# Autodesk Inventor assembly: Joes_Robot
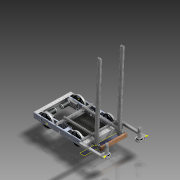
[picture p0: Inventor's stored thumbnail of the model, 180x180]
Saved by Autodesk Inventor 2015 (Build 190159000, 159)
## iProperties
Created: 2015-01-23
Part Number: Joes_Robot
Document SubType Name: Assembly
Designer: 55221
Author: 55221
## Documents named in this file (27)
- C:\Users\Kingbob26\Documents\GitHub\2015CAD\Misc\Joes_Robot.iam
- C:\Users\Kingbob26\Documents\GitHub\2015CAD\wheelBase\Outside Sheet Square.ipt
- C:\Users\Kingbob26\Documents\GitHub\2015CAD\wheelBase\2x3 Hole Bracket.ipt
- C:\Users\Kingbob26\Documents\GitHub\2015CAD\wheelBase\Inside Sheet Square.ipt
- C:\Users\Kingbob26\Documents\GitHub\2015CAD\wheelBase\TB Output Shaft Hex L-Base 2.ipt
- C:\Users\Kingbob26\Documents\Inventor\Sheet Metal Front-Back.ipt.ipt
- C:\Users\Kingbob26\Documents\GitHub\2015CAD\actualWheelBase\Drive Base\Parts\simpleGBFull.iam
- C:\Users\Kingbob26\Documents\GitHub\2015CAD\actualWheelBase\Drive Base\Parts\8inDriveWheel.iam
- C:\Users\Kingbob26\Documents\GitHub\2015CAD\wheelBase\Hex Bearing.ipt
- C:\Users\Kingbob26\Documents\GitHub\2015CAD\Motion\alignmentWheelsBar.ipt
- C:\Users\Kingbob26\Documents\GitHub\2015CAD\Motion\alignmentWheelsBarP2.ipt
- C:\Users\Kingbob26\Documents\GitHub\2015CAD\Motion\alignmentWheelsMotor.ipt
- C:\Users\Kingbob26\Documents\GitHub\2015CAD\wheelBase\4in 2013 Hub.ipt
- C:\Users\Kingbob26\Documents\GitHub\2015CAD\wheelBase\4 in tread.ipt
- C:\Users\Kingbob26\Documents\GitHub\2015CAD\wheelBase\keyStoneHub10mm.ipt
- C:\Users\Kingbob26\Documents\GitHub\2015CAD\Misc\Imported Components\T-slottedFraming\T-slottedFraming.ipt
- C:\Users\Kingbob26\Documents\GitHub\2015CAD\Motion\GuidanceShaft.ipt
- C:\Users\Kingbob26\Documents\GitHub\2015CAD\Motion\Roller.ipt
- C:\Users\Kingbob26\Documents\GitHub\2015CAD\Misc\Imported Components\90framing\90framing.ipt
- C:\Users\Kingbob26\Documents\GitHub\2015CAD\Misc\Imported Components\specialScrews\specialScrews.ipt
- C:\Users\Kingbob26\Documents\GitHub\2015CAD\Misc\T-slottedFramingCustomLength25.5.ipt
- C:\Users\Kingbob26\Documents\GitHub\2015CAD\Misc\Imported Components\90degreeAngleBracket\90degreeAngleBracket.ipt
- C:\Users\Kingbob26\Documents\GitHub\2015CAD\Misc\liftingMechanismPlate.ipt
- C:\Users\Kingbob26\Documents\GitHub\2015CAD\Misc\Imported Components\1x1tCap\1x1tCap.ipt
- C:\Users\Kingbob26\Documents\GitHub\2015CAD\Misc\Crossbar.ipt
- C:\Users\Kingbob26\Documents\GitHub\2015CAD\Motion\lBracketForLiftingBar.ipt
- Sheet Metal Front-Back.ipt
## Components (60 placed, 25 different names)
1. Outside Sheet Square:1 — Mate:124, Mate:181, Mate:183, Mate:189, Mate:206, Mate:207, Mate:245, Mate:246, Mate:335
2. 2x3 Hole Bracket:2 — Mate:116, Mate:117, Mate:118, Mate:124, Mate:335
3. Inside Sheet Square:1 — Mate:116, Mate:117, Mate:118, Mate:150, Mate:182, Mate:184, Mate:188, Mate:204, Mate:205, Angle:9, Flush:2
4. Inside Sheet Square:2 — Mate:131, Mate:132, Mate:134, Mate:180, Mate:185, Insert:1, Angle:5, Mate:201, Mate:202, Mate:203, Flush:3, Mate:316, Mate:317, Mate:318
5. Outside Sheet Square:2 — Mate:133, Mate:178, Mate:179, Mate:186, Mate:187, Mate:208, Mate:209, Mate:247, Mate:248, Mate:263, Mate:281, Mate:298, Mate:300
6. 2x3 Hole Bracket:3 — Mate:131, Mate:132, Mate:133, Mate:134, Mate:281
7. TB Output Shaft Hex L-Base 2:3 — Mate:150, Angle:8
8. Sheet Metal Front-Back.ipt:1 — Mate:178, Mate:179, Mate:180, Mate:181, Mate:182, Mate:183, Mate:184, Angle:17, Mate:278, Mate:282, Flush:4, Mate:299, Flush:8, Mate:303, Flush:19, Flush:22
9. Sheet Metal Front-Back.ipt:2 — Mate:185, Mate:186, Mate:187, Mate:188, Mate:189, Mate:263
10. simpleGBFull:1 [sub-assembly] — Angle:9
11. 8inDriveWheel:1 [sub-assembly]
12. simpleGBFull:2 [sub-assembly] — Insert:1, Angle:5, Mate:198, Mate:199
13. TB Output Shaft Hex L-Base 2:4 — Mate:198, Mate:199, Mate:200, Angle:6, Angle:7
14. 8inDriveWheel:4 [sub-assembly] — Mate:200, Angle:6, Mate:201
15. 8inDriveWheel:5 [sub-assembly] — Mate:202, Mate:203
16. 8inDriveWheel:6 [sub-assembly] — Mate:204, Mate:205
17. Hex Bearing:1 — Mate:206, Mate:207, Angle:8
18. Hex Bearing:2 — Mate:208, Mate:209, Angle:7
19. alignmentWheelsBar:1 — Mate:217, Mate:218, Mate:245, Mate:246
20. alignmentWheelsBar:2 — Mate:243, Mate:244, Mate:247, Mate:248
21. alignmentWheelsBarP2:1 — Mate:243, Mate:244, Insert:4, Mate:251
22. alignmentWheelsBarP2:2 — Mate:217, Mate:218, Insert:5, Mate:249
23. alignmentWheelsMotor:1 — Angle:10, Mate:249, Mate:250
24. alignmentWheelsMotor:2 — Angle:11, Mate:251, Mate:252
25. 4in 2013 Hub:1 — Insert:3, Mate:237, Mate:238, Mate:239
26. 4in 2013 Hub:2 — Insert:2, Mate:240, Mate:241, Mate:242
27. 4 in tread:1 — Insert:3
28. 4 in tread:2 — Insert:2
29. keyStoneHub10mm:1 — Mate:237, Mate:238, Mate:239, Angle:10, Insert:5, Mate:250
30. keyStoneHub10mm:2 — Mate:240, Mate:241, Mate:242, Angle:11, Insert:4, Mate:252
31. T-slottedFraming:1 — Flush:4, Mate:291, Mate:296, Mate:298, Mate:299, Flush:9, Mate:301, Mate:305, Mate:306, Mate:308, Flush:18
32. GuidanceShaft:1 — Flush:2, Angle:17, Mate:278, Mate:279, Mate:280, Angle:20, Angle:21, Angle:22, Angle:28, Angle:29, Mate:321, Mate:322
33. GuidanceShaft:2 — Flush:3, Mate:271, Mate:282
34. Roller:1 — Angle:28, Angle:29, Mate:321, Mate:322, Mate:324, Mate:325, Mate:326, Angle:30, Mate:329, Flush:20, Flush:21
35. 90framing:1 — Mate:271, Insert:6, Angle:13, Angle:14, Insert:7, Mate:320, Flush:17
36. specialScrews:1 — Insert:6, Angle:13
37. specialScrews:3 — Angle:14, Insert:7
38. 90framing:2 — Mate:279, Mate:280, Insert:8, Insert:9, Mate:319, Flush:16
39. T-slottedFraming:2 — Mate:288, Mate:292, Flush:5, Mate:294, Mate:300, Flush:8, Mate:303, Angle:23, Mate:304, Flush:11, Mate:310, Mate:312
40. specialScrews:4 — Angle:20, Insert:8
41. specialScrews:5 — Angle:21, Insert:9
42. T-slottedFramingCustomLength25.5:1 — Mate:288, Angle:22, Mate:291, Flush:5, Mate:293, Flush:6, Mate:295, Mate:297, Mate:302, Mate:320, Flush:17, Angle:24, Insert:10, Angle:26, Insert:12, Flush:18
43. T-slottedFramingCustomLength25.5:2 — Angle:23, Mate:304, Flush:11, Mate:305, Mate:307, Mate:309, Mate:311, Mate:313, Mate:319, Flush:16, Angle:25, Insert:11, Angle:27, Insert:13, Flush:19
44. 90degreeAngleBracket:1 — Mate:294, Mate:295, Flush:7, Flush:14
45. 90degreeAngleBracket:2 — Mate:301, Mate:302, Flush:10, Flush:12
46. 90degreeAngleBracket:3 — Mate:296, Mate:297, Flush:9, Flush:10, Flush:13
47. 90degreeAngleBracket:4 — Mate:292, Mate:293, Flush:6, Flush:7
48. 90degreeAngleBracket:5 — Mate:308, Mate:309, Flush:13
49. 90degreeAngleBracket:6 — Mate:306, Mate:307, Flush:12
50. 90degreeAngleBracket:7 — Mate:312, Mate:313, Flush:15
51. 90degreeAngleBracket:8 — Mate:310, Mate:311, Flush:14, Flush:15
52. liftingMechanismPlate:1 — Mate:316, Mate:317, Mate:318
53. 1x1tCap:1 — Angle:27, Insert:13
54. 1x1tCap:2 — Angle:26, Insert:12
55. 1x1tCap:3 — Angle:25, Insert:11
56. 1x1tCap:4 — Angle:24, Insert:10
57. Crossbar:1 — Mate:328, Mate:333, Mate:334
58. Roller:2 — Angle:30, Mate:329, Flush:20, Flush:21, Mate:330, Mate:331, Mate:332
59. lBracketForLiftingBar:1 — Mate:324, Mate:325, Mate:326, Mate:328, Mate:333, Mate:334
60. lBracketForLiftingBar:3 — Mate:330, Mate:331, Mate:332
## Relationships (161: Mate 106, Angle 21, Flush 21, Insert 13)
- [Mate]: TB Output Shaft Hex L-Base 2:3 ↔ simpleGBFull:1
- Mate:116: 2x3 Hole Bracket:2 ↔ Inside Sheet Square:1
- Mate:117: 2x3 Hole Bracket:2 ↔ Inside Sheet Square:1
- Mate:118: 2x3 Hole Bracket:2 ↔ Inside Sheet Square:1
- Mate:124: Outside Sheet Square:1 ↔ 2x3 Hole Bracket:2
- Mate:131: Inside Sheet Square:2 ↔ 2x3 Hole Bracket:3
- Mate:132: Inside Sheet Square:2 ↔ 2x3 Hole Bracket:3
- Mate:133: Outside Sheet Square:2 ↔ 2x3 Hole Bracket:3
- Mate:134: Inside Sheet Square:2 ↔ 2x3 Hole Bracket:3
- [Mate]: Inside Sheet Square:1 ↔ simpleGBFull:1
- Mate:150: Inside Sheet Square:1 ↔ TB Output Shaft Hex L-Base 2:3
- [Mate]: TB Output Shaft Hex L-Base 2:3 ↔ simpleGBFull:1
- Mate:178: Outside Sheet Square:2 ↔ Sheet Metal Front-Back.ipt:1
- Mate:179: Outside Sheet Square:2 ↔ Sheet Metal Front-Back.ipt:1
- Mate:180: Inside Sheet Square:2 ↔ Sheet Metal Front-Back.ipt:1
- Mate:181: Outside Sheet Square:1 ↔ Sheet Metal Front-Back.ipt:1
- Mate:182: Inside Sheet Square:1 ↔ Sheet Metal Front-Back.ipt:1
- Mate:183: Outside Sheet Square:1 ↔ Sheet Metal Front-Back.ipt:1
- Mate:184: Inside Sheet Square:1 ↔ Sheet Metal Front-Back.ipt:1
- Mate:185: Inside Sheet Square:2 ↔ Sheet Metal Front-Back.ipt:2
- Mate:186: Outside Sheet Square:2 ↔ Sheet Metal Front-Back.ipt:2
- Mate:187: Outside Sheet Square:2 ↔ Sheet Metal Front-Back.ipt:2
- Mate:188: Inside Sheet Square:1 ↔ Sheet Metal Front-Back.ipt:2
- Mate:189: Outside Sheet Square:1 ↔ Sheet Metal Front-Back.ipt:2
- [Mate]: TB Output Shaft Hex L-Base 2:3 ↔ 8inDriveWheel:1
- [Mate]: TB Output Shaft Hex L-Base 2:3 ↔ 8inDriveWheel:1
- [Mate]: Inside Sheet Square:1 ↔ 8inDriveWheel:1
- Insert:1: Inside Sheet Square:2 ↔ simpleGBFull:2
- Angle:5 (0 deg): Inside Sheet Square:2 ↔ simpleGBFull:2
- Mate:198: simpleGBFull:2 ↔ TB Output Shaft Hex L-Base 2:4
- Mate:199: simpleGBFull:2 ↔ TB Output Shaft Hex L-Base 2:4
- Mate:200: TB Output Shaft Hex L-Base 2:4 ↔ 8inDriveWheel:4
- Angle:6 (0 deg): TB Output Shaft Hex L-Base 2:4 ↔ 8inDriveWheel:4
- Mate:201: Inside Sheet Square:2 ↔ 8inDriveWheel:4
- Mate:202: Inside Sheet Square:2 ↔ 8inDriveWheel:5
- Mate:203: Inside Sheet Square:2 ↔ 8inDriveWheel:5
- Mate:204: Inside Sheet Square:1 ↔ 8inDriveWheel:6
- Mate:205: Inside Sheet Square:1 ↔ 8inDriveWheel:6
- Mate:206: Outside Sheet Square:1 ↔ Hex Bearing:1
- Mate:207: Outside Sheet Square:1 ↔ Hex Bearing:1
- Mate:208: Outside Sheet Square:2 ↔ Hex Bearing:2
- Mate:209: Outside Sheet Square:2 ↔ Hex Bearing:2
- Angle:7 (0 deg): TB Output Shaft Hex L-Base 2:4 ↔ Hex Bearing:2
- Angle:8 (0 deg): TB Output Shaft Hex L-Base 2:3 ↔ Hex Bearing:1
- Angle:9 (0 deg): Inside Sheet Square:1 ↔ simpleGBFull:1
- Mate:217: alignmentWheelsBar:1 ↔ alignmentWheelsBarP2:2
- Mate:218: alignmentWheelsBar:1 ↔ alignmentWheelsBarP2:2
- Insert:2: 4in 2013 Hub:2 ↔ 4 in tread:2
- Insert:3: 4in 2013 Hub:1 ↔ 4 in tread:1
- Mate:237: 4in 2013 Hub:1 ↔ keyStoneHub10mm:1
- Mate:238: 4in 2013 Hub:1 ↔ keyStoneHub10mm:1
- Mate:239: 4in 2013 Hub:1 ↔ keyStoneHub10mm:1
- Mate:240: 4in 2013 Hub:2 ↔ keyStoneHub10mm:2
- Mate:241: 4in 2013 Hub:2 ↔ keyStoneHub10mm:2
- Mate:242: 4in 2013 Hub:2 ↔ keyStoneHub10mm:2
- Angle:10 (0 deg): alignmentWheelsMotor:1 ↔ keyStoneHub10mm:1
- Angle:11 (180 deg): alignmentWheelsMotor:2 ↔ keyStoneHub10mm:2
- Mate:243: alignmentWheelsBar:2 ↔ alignmentWheelsBarP2:1
- Mate:244: alignmentWheelsBar:2 ↔ alignmentWheelsBarP2:1
- Mate:245 (19.0754 mm): Outside Sheet Square:1 ↔ alignmentWheelsBar:1
- Mate:246: Outside Sheet Square:1 ↔ alignmentWheelsBar:1
- Mate:247 (19.0754 mm): Outside Sheet Square:2 ↔ alignmentWheelsBar:2
- Mate:248: Outside Sheet Square:2 ↔ alignmentWheelsBar:2
- Insert:4: alignmentWheelsBarP2:1 ↔ keyStoneHub10mm:2
- Insert:5: alignmentWheelsBarP2:2 ↔ keyStoneHub10mm:1
- Mate:249: alignmentWheelsBarP2:2 ↔ alignmentWheelsMotor:1
- Mate:250: alignmentWheelsMotor:1 ↔ keyStoneHub10mm:1
- Mate:251: alignmentWheelsBarP2:1 ↔ alignmentWheelsMotor:2
- Mate:252: alignmentWheelsMotor:2 ↔ keyStoneHub10mm:2
- Mate:263: Outside Sheet Square:2 ↔ Sheet Metal Front-Back.ipt:2
- Flush:2: Inside Sheet Square:1 ↔ GuidanceShaft:1
- Flush:3: Inside Sheet Square:2 ↔ GuidanceShaft:2
- Mate:271: GuidanceShaft:2 ↔ 90framing:1
- Insert:6: 90framing:1 ↔ specialScrews:1
- Angle:13 (0 deg): 90framing:1 ↔ specialScrews:1
- Angle:14 (0 deg): 90framing:1 ↔ specialScrews:3
- Insert:7: 90framing:1 ↔ specialScrews:3
- Angle:17 (0 deg): Sheet Metal Front-Back.ipt:1 ↔ GuidanceShaft:1
- Mate:278 (38.1 mm): Sheet Metal Front-Back.ipt:1 ↔ GuidanceShaft:1
- Mate:279 (2.54 mm): GuidanceShaft:1 ↔ 90framing:2
- Mate:280: GuidanceShaft:1 ↔ 90framing:2
- Mate:281: Outside Sheet Square:2 ↔ 2x3 Hole Bracket:3
- Mate:282 (38.1 mm): Sheet Metal Front-Back.ipt:1 ↔ GuidanceShaft:2
- Angle:20 (0 deg): GuidanceShaft:1 ↔ specialScrews:4
- Angle:21 (0 deg): GuidanceShaft:1 ↔ specialScrews:5
- Insert:8: 90framing:2 ↔ specialScrews:4
- Insert:9: 90framing:2 ↔ specialScrews:5
- Mate:288 (16.256 mm): T-slottedFraming:2 ↔ T-slottedFramingCustomLength25.5:1
- Angle:22 (0 deg): GuidanceShaft:1 ↔ T-slottedFramingCustomLength25.5:1
- Flush:4: Sheet Metal Front-Back.ipt:1 ↔ T-slottedFraming:1
- Mate:291 (16.256 mm): T-slottedFraming:1 ↔ T-slottedFramingCustomLength25.5:1
- Mate:292 (8.128 mm): T-slottedFraming:2 ↔ 90degreeAngleBracket:4
- Flush:5 (-8.128 mm): T-slottedFraming:2 ↔ T-slottedFramingCustomLength25.5:1
- Mate:293 (8.128 mm): T-slottedFramingCustomLength25.5:1 ↔ 90degreeAngleBracket:4
- Flush:6 (3.683 mm): T-slottedFramingCustomLength25.5:1 ↔ 90degreeAngleBracket:4
- Mate:294 (8.128 mm): T-slottedFraming:2 ↔ 90degreeAngleBracket:1
- Mate:295 (8.128 mm): T-slottedFramingCustomLength25.5:1 ↔ 90degreeAngleBracket:1
- Flush:7: 90degreeAngleBracket:1 ↔ 90degreeAngleBracket:4
- Mate:296 (8.128 mm): T-slottedFraming:1 ↔ 90degreeAngleBracket:3
- Mate:297 (8.128 mm): T-slottedFramingCustomLength25.5:1 ↔ 90degreeAngleBracket:3
- Mate:298 (8.128 mm): Outside Sheet Square:2 ↔ T-slottedFraming:1
- Mate:299 (8.128 mm): Sheet Metal Front-Back.ipt:1 ↔ T-slottedFraming:1
- Mate:300 (8.128 mm): Outside Sheet Square:2 ↔ T-slottedFraming:2
- Flush:8: Sheet Metal Front-Back.ipt:1 ↔ T-slottedFraming:2
- Flush:9 (-4.445 mm): T-slottedFraming:1 ↔ 90degreeAngleBracket:3
- Mate:301 (8.128 mm): T-slottedFraming:1 ↔ 90degreeAngleBracket:2
- Mate:302 (8.128 mm): T-slottedFramingCustomLength25.5:1 ↔ 90degreeAngleBracket:2
- Flush:10: 90degreeAngleBracket:2 ↔ 90degreeAngleBracket:3
- Mate:303 (415.544 mm): Sheet Metal Front-Back.ipt:1 ↔ T-slottedFraming:2
- Angle:23 (0 deg): T-slottedFraming:2 ↔ T-slottedFramingCustomLength25.5:2
- Mate:304 (16.256 mm): T-slottedFraming:2 ↔ T-slottedFramingCustomLength25.5:2
- Flush:11 (-8.128 mm): T-slottedFraming:2 ↔ T-slottedFramingCustomLength25.5:2
- Mate:305 (16.256 mm): T-slottedFraming:1 ↔ T-slottedFramingCustomLength25.5:2
- Mate:306 (8.128 mm): T-slottedFraming:1 ↔ 90degreeAngleBracket:6
- Mate:307 (8.128 mm): T-slottedFramingCustomLength25.5:2 ↔ 90degreeAngleBracket:6
- Flush:12: 90degreeAngleBracket:2 ↔ 90degreeAngleBracket:6
- Mate:308 (8.128 mm): T-slottedFraming:1 ↔ 90degreeAngleBracket:5
- Mate:309 (8.128 mm): T-slottedFramingCustomLength25.5:2 ↔ 90degreeAngleBracket:5
- Flush:13: 90degreeAngleBracket:3 ↔ 90degreeAngleBracket:5
- Mate:310 (8.128 mm): T-slottedFraming:2 ↔ 90degreeAngleBracket:8
- Mate:311 (8.128 mm): T-slottedFramingCustomLength25.5:2 ↔ 90degreeAngleBracket:8
- Flush:14: 90degreeAngleBracket:1 ↔ 90degreeAngleBracket:8
- Mate:312 (8.128 mm): T-slottedFraming:2 ↔ 90degreeAngleBracket:7
- Mate:313 (8.128 mm): T-slottedFramingCustomLength25.5:2 ↔ 90degreeAngleBracket:7
- Flush:15: 90degreeAngleBracket:7 ↔ 90degreeAngleBracket:8
- Mate:316: Inside Sheet Square:2 ↔ liftingMechanismPlate:1
- Mate:317: Inside Sheet Square:2 ↔ liftingMechanismPlate:1
- Mate:318: Inside Sheet Square:2 ↔ liftingMechanismPlate:1
- Mate:319 (8.128 mm): 90framing:2 ↔ T-slottedFramingCustomLength25.5:2
- Flush:16 (-8.128 mm): 90framing:2 ↔ T-slottedFramingCustomLength25.5:2
- Mate:320 (8.128 mm): 90framing:1 ↔ T-slottedFramingCustomLength25.5:1
- Flush:17 (-8.128 mm): 90framing:1 ↔ T-slottedFramingCustomLength25.5:1
- Angle:24 (0 deg): T-slottedFramingCustomLength25.5:1 ↔ 1x1tCap:4
- Insert:10: T-slottedFramingCustomLength25.5:1 ↔ 1x1tCap:4
- Angle:25 (0 deg): T-slottedFramingCustomLength25.5:2 ↔ 1x1tCap:3
- Insert:11: T-slottedFramingCustomLength25.5:2 ↔ 1x1tCap:3
- Angle:26 (0 deg): T-slottedFramingCustomLength25.5:1 ↔ 1x1tCap:2
- Angle:27 (0 deg): T-slottedFramingCustomLength25.5:2 ↔ 1x1tCap:1
- Insert:12: T-slottedFramingCustomLength25.5:1 ↔ 1x1tCap:2
- Insert:13: T-slottedFramingCustomLength25.5:2 ↔ 1x1tCap:1
- Flush:18 (135.128 mm): T-slottedFraming:1 ↔ T-slottedFramingCustomLength25.5:1
- Angle:28 (0 deg): GuidanceShaft:1 ↔ Roller:1
- Angle:29 (0 deg): GuidanceShaft:1 ↔ Roller:1
- Mate:321 (22.606 mm): GuidanceShaft:1 ↔ Roller:1
- Mate:322 (11.684 mm): GuidanceShaft:1 ↔ Roller:1
- Flush:19 (135.128 mm): Sheet Metal Front-Back.ipt:1 ↔ T-slottedFramingCustomLength25.5:2
- Mate:324: Roller:1 ↔ lBracketForLiftingBar:1
- Mate:325: Roller:1 ↔ lBracketForLiftingBar:1
- Mate:326: Roller:1 ↔ lBracketForLiftingBar:1
- Mate:328: Crossbar:1 ↔ lBracketForLiftingBar:1
- Angle:30 (0 deg): Roller:1 ↔ Roller:2
- Mate:329 (384.81 mm): Roller:1 ↔ Roller:2
- Flush:20: Roller:1 ↔ Roller:2
- Flush:21: Roller:1 ↔ Roller:2
- Mate:330: Roller:2 ↔ lBracketForLiftingBar:3
- Mate:331: Roller:2 ↔ lBracketForLiftingBar:3
- Mate:332: Roller:2 ↔ lBracketForLiftingBar:3
- Mate:333: Crossbar:1 ↔ lBracketForLiftingBar:1
- Mate:334: Crossbar:1 ↔ lBracketForLiftingBar:1
- Mate:335: Outside Sheet Square:1 ↔ 2x3 Hole Bracket:2
- Flush:22 (63.5 mm): Sheet Metal Front-Back.ipt:1
